# Autodesk Inventor assembly: side guard
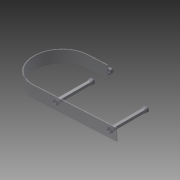
[picture p0: Inventor's stored thumbnail of the model, 180x180]
Saved by Autodesk Inventor 2014 SP1 (Build 180222100, 222)
## iProperties
Created: 2013-11-11
Part Number: side guard
Document SubType Name: Assembly
Designer: RyanHughes
Author: RyanHughes
## Documents named in this file (5)
- C:\Users\Ryan\Desktop\sw\toss up 2ed A bot\intake\side guard.iam
- C:\Users\Ryan\Desktop\sw\lib\Aperture VEX CAD Library\Hardware\8-32\8-32 Nylock.ipt
- C:\Users\Ryan\Desktop\sw\lib\Aperture VEX CAD Library\Standoffs\BEAM-2000.ipt
- C:\Users\Ryan\Desktop\sw\lib\Aperture VEX CAD Library\Metal\C Channel\2 x 8.ipt
- C:\Users\Ryan\Desktop\sw\toss up 2ed A bot\intake\buckies poly\side guard.ipt
## Components (9 placed, 4 different names)
1. 2 x 8:1 — Mate:5, Mate:6, Mate:7, Angle:1, Mate:12, Mate:13
2. side guard:1 — Angle:1, Mate:8, Mate:9, Mate:10, Mate:11
3. 8-32 Nylock:5 — Mate:11, Mate:12, Mate:13
4. 8-32 Nylock:1 — Mate:6, Mate:7
5. BEAM-2000:1 — Mate:9
6. 8-32 Nylock:2 — Mate:5
7. 8-32 Nylock:3 — Mate:8, Mate:10
8. BEAM-2000:2
9. 8-32 Nylock:4
## Component patterns: (2 elements, first: 8-32 Nylock:1 + BEAM-2000:1 + 8-32 Nylock:2)
## Relationships (14: Mate 13, Angle 1)
- [Mate]: 8-32 Nylock:1 ↔ BEAM-2000:1
- [Mate]: 8-32 Nylock:1 ↔ BEAM-2000:1
- [Mate]: BEAM-2000:1 ↔ 8-32 Nylock:2
- [Mate]: BEAM-2000:1 ↔ 8-32 Nylock:2
- Mate:5: 2 x 8:1 ↔ 8-32 Nylock:2
- Mate:6 (2.3114 mm): 2 x 8:1 ↔ 8-32 Nylock:1
- Mate:7 (2.3114 mm): 2 x 8:1 ↔ 8-32 Nylock:1
- Angle:1 (0 deg): 2 x 8:1 ↔ side guard:1
- Mate:8: side guard:1 ↔ 8-32 Nylock:3
- Mate:9: side guard:1 ↔ BEAM-2000:1
- Mate:10: side guard:1 ↔ 8-32 Nylock:3
- Mate:11: side guard:1 ↔ 8-32 Nylock:5
- Mate:12 (2.3114 mm): 2 x 8:1 ↔ 8-32 Nylock:5
- Mate:13 (2.3114 mm): 2 x 8:1 ↔ 8-32 Nylock:5
## Named parameters: q = 2.3114 mm
